# Autodesk Inventor assembly: Assembly
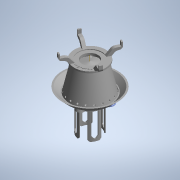
[picture p0: Inventor's stored thumbnail of the model, 180x180]
Saved by Autodesk Inventor 2022.4 (Build 264492010, 492A)
## iProperties
Part Number: Assembly
Document SubType Name: Assembly
Designer: tmass
Author: tmass
## Documents named in this file (5)
- C:\Users\tmass\OneDrive\Bureau\UFO paper\3D models\UFO\Inventor\Assembly.iam
- C:\Users\tmass\OneDrive\Bureau\UFO paper\3D models\UFO\Inventor\Box.ipt
- C:\Users\tmass\OneDrive\Bureau\UFO paper\3D models\UFO\Inventor\Top cover 4 vials.ipt
- C:\Users\tmass\OneDrive\Bureau\UFO paper\3D models\UFO\Inventor\bottom part Heidolf adaptor.ipt
- C:\Users\tmass\OneDrive\Bureau\UFO paper\3D models\UFO\Inventor\Reflector final.ipt
## Components (4 placed, 4 different names)
1. Box:1 — Mate:1, Mate:2, Mate:3, Mate:5, Mate:6
2. Top cover 4 vials:1 — Mate:1, Mate:6
3. bottom part Heidolf adaptor:1 — Mate:3, Mate:4, Mate:5
4. Reflector final:1 — Mate:2, Mate:4
## Relationships (6: Mate 6)
- Mate:1: Box:1 ↔ Top cover 4 vials:1
- Mate:2: Box:1 ↔ Reflector final:1
- Mate:3: Box:1 ↔ bottom part Heidolf adaptor:1
- Mate:4: bottom part Heidolf adaptor:1 ↔ Reflector final:1
- Mate:5: Box:1 ↔ bottom part Heidolf adaptor:1
- Mate:6: Box:1 ↔ Top cover 4 vials:1
